# Autodesk Inventor assembly: BetterModel
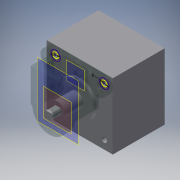
[picture p0: Inventor's stored thumbnail of the model, 180x180]
Saved by Autodesk Inventor 2019 (Build 230136000, 136)
## iProperties
Created: 2021-03-26
Part Number: BetterModel
Document SubType Name: Assembly
Designer: Ian
Author: Ian
## Documents named in this file (10)
- D:\Ian\Documents\Projects\PiHome\3D Models\Update\BetterModel.iam
- D:\Ian\Documents\Projects\PiHome\3D Models\Update\stepper.ipt
- D:\Ian\Documents\Projects\PiHome\3D Models\Update\big one.ipt
- D:\Ian\Documents\Projects\PiHome\3D Models\Update\Bracket.ipt
- D:\Ian\Documents\Projects\PiHome\3D Models\Update\smaller.ipt
- D:\Users\Ian\Downloads\TPU Pad.ipt
- D:\Ian\Documents\Projects\PiHome\3D Models\Update\Shelf.ipt
- D:\Ian\Documents\Projects\PiHome\3D Models\Update\Shelf Braket.ipt
- D:\Ian\Documents\Projects\PiHome\3D Models\Update\tpu pad 2.ipt
- D:\Ian\Documents\Projects\Big Printer\X-Axis Temp Redesign November 2021\STLs\newDriveWheel.ipt
## Components (9 placed, 9 different names)
1. stepper:1 — Flush:1, Flush:2, Flush:5, Flush:8, Flush:12, Flush:13
2. big one:1 — Flush:1, Flush:2, Flush:3, Flush:4, Flush:6
3. smaller:1 — Flush:5, Flush:6, Flush:7
4. Bracket:1 — Flush:3, Flush:4, Flush:7, Flush:16
5. TPU Pad:1 — Flush:8, Flush:10, Flush:11
6. Shelf:1 — Flush:10, Flush:11
7. Shelf Braket:1 — Flush:12, Flush:13, Flush:14, Flush:15
8. tpu pad 2:1 — Flush:14, Flush:15
9. newDriveWheel:1 — Flush:16
## Relationships (15: Flush 15)
- Flush:1: stepper:1 ↔ big one:1
- Flush:2 (0.1 mm): stepper:1 ↔ big one:1
- Flush:3: big one:1 ↔ Bracket:1
- Flush:4 (0.1 mm): big one:1 ↔ Bracket:1
- Flush:5: stepper:1 ↔ smaller:1
- Flush:6: big one:1 ↔ smaller:1
- Flush:7 (0.1 mm): smaller:1 ↔ Bracket:1
- Flush:8: stepper:1 ↔ TPU Pad:1
- Flush:10: TPU Pad:1 ↔ Shelf:1
- Flush:11: TPU Pad:1 ↔ Shelf:1
- Flush:12: stepper:1 ↔ Shelf Braket:1
- Flush:13: stepper:1 ↔ Shelf Braket:1
- Flush:14: Shelf Braket:1 ↔ tpu pad 2:1
- Flush:15: Shelf Braket:1 ↔ tpu pad 2:1
- Flush:16 (0.2 mm): Bracket:1 ↔ newDriveWheel:1
